# Autodesk Inventor assembly: Protocube
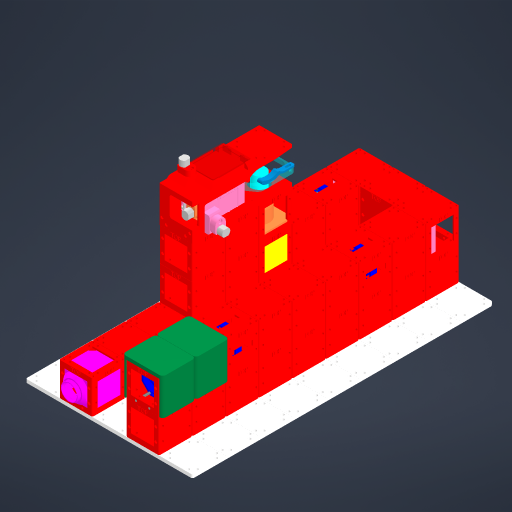
[picture p0: Inventor's stored thumbnail of the model, 512x512]
Saved by Autodesk Inventor 2023.4 (Build 274418000, 418)
## iProperties
Created: 2022-08-13
Part Number: Protocube
Document SubType Name: Assembly
Designer: xSibe
Author: xSibe
## Documents named in this file (12)
- C:\.Laptop\.Work\Projects\Project Protocube\Github\CAD, STL, OBJ Files\1 CAD\Protocube.iam
- C:\.Laptop\.Work\Projects\Project Protocube\1 Autodesk\1 Cubes\Baseplates\Baseplate 9x5 V5.ipt
- C:\.Laptop\.Work\Projects\Project Protocube\1 Autodesk\1 Cubes\Laser\Cube 1x1 V5 (Green Laser).iam
- C:\.Laptop\.Work\Projects\Project Protocube\1 Autodesk\1 Cubes\Lense\Cube 1x1 V5 (Half Inch Lense).iam
- C:\.Laptop\.Work\Projects\Project Protocube\1 Autodesk\1 Cubes\Mirror\Cube 1x1 V5 (Mirror Vertical).iam
- C:\.Laptop\.Work\Projects\Project Protocube\1 Autodesk\1 Cubes\Dichroic\Cube 1x1 V5 (Dichroic).iam
- C:\.Laptop\.Work\Projects\Project Protocube\1 Autodesk\1 Cubes\Objective\Cube 1x1 V5 (Objective).iam
- C:\.Laptop\.Work\Projects\Project Protocube\1 Autodesk\1 Cubes\Camera\Cube 1x1 V5 (Camera).iam
- C:\.Laptop\.Work\Projects\Project Protocube\1 Autodesk\1 Cubes\Mirror\Cube 1x1 V5 (Mirror Horizontal).iam
- C:\.Laptop\.Work\Projects\Project Protocube\1 Autodesk\1 Cubes\Cubes\Cube 1x1 V5 Closed.iam
- C:\.Laptop\.Work\Projects\Project Protocube\1 Autodesk\1 Cubes\Lense\Cube 1x1 V5 (One Inch Lense).iam
- C:\.Laptop\.Work\Projects\Project Protocube\1 Autodesk\1 Cubes\XYZ Stage\XYZ Stage V5.iam
## Components (39 placed, 11 different names)
1. Baseplate 9x5 V5:1 — Mate:27, Mate:46, Mate:47, Mate:48, Mate:52, Mate:53, Mate:60, Mate:61, Mate:62, Mate:65, Mate:66, Mate:67, Mate:69, Mate:70, Mate:71, Mate:93, Mate:94, Mate:95, Mate:98, Mate:99, Mate:100
2. Cube 1x1 V5 (Green Laser):1 [sub-assembly] — Mate:76, Flush:6, Flush:7
3. Cube 1x1 V5 (Mirror Vertical):1 [sub-assembly] — Mate:46, Mate:47, Mate:48, Flush:22, Flush:86, Mate:92
4. Cube 1x1 V5 (Mirror Horizontal):1 [sub-assembly] — Mate:81, Flush:14, Flush:15
5. Cube 1x1 V5 (Mirror Horizontal):2 [sub-assembly] — Flush:16, Flush:17, Mate:82
6. Cube 1x1 V5 (Half Inch Lense):1 [sub-assembly] — Mate:77, Flush:8, Flush:9
7. Cube 1x1 V5 (One Inch Lense):1 [sub-assembly] — Mate:96, Flush:87, Flush:88
8. Cube 1x1 V5 (One Inch Lense):2 [sub-assembly] — Mate:97, Flush:89, Flush:90
9. Cube 1x1 V5 (One Inch Lense):3 [sub-assembly] — Mate:98, Mate:99, Mate:100
10. Cube 1x1 V5 (Dichroic):1 [sub-assembly] — Flush:22, Flush:86, Mate:86, Flush:23, Flush:24, Mate:92
11. Cube 1x1 V5 (Camera):1 [sub-assembly] — Mate:27, Mate:52, Mate:53
12. Cube 1x1 V5 (Objective):1 [sub-assembly] — Mate:86, Flush:23, Flush:24, Mate:101, Mate:102, Mate:103
13. XYZ Stage V5:1 [sub-assembly] — Mate:101, Mate:102, Mate:103
14. Cube 1x1 V5 Closed:13 [sub-assembly] — Flush:3, Mate:80, Flush:13
15. Cube 1x1 V5 Closed:17 [sub-assembly] — Flush:20, Flush:21, Mate:84
16. Cube 1x1 V5 Closed:1 [sub-assembly] — Mate:60, Mate:61, Mate:62, Mate:76, Flush:6, Flush:7
17. Cube 1x1 V5 Closed:2 [sub-assembly]
18. Cube 1x1 V5 Closed:3 [sub-assembly] — Mate:77, Flush:8, Flush:9
19. Cube 1x1 V5 Closed:4 [sub-assembly] — Flush:2, Mate:78, Flush:10
20. Cube 1x1 V5 Closed:5 [sub-assembly]
21. Cube 1x1 V5 Closed:6 [sub-assembly]
22. Cube 1x1 V5 Closed:7 [sub-assembly] — Mate:96, Flush:87, Flush:88
23. Cube 1x1 V5 Closed:8 [sub-assembly] — Flush:3, Mate:80, Flush:13
24. Cube 1x1 V5 Closed:9 [sub-assembly] — Mate:81, Flush:14, Flush:15
25. Cube 1x1 V5 Closed:10 [sub-assembly] — Flush:2, Mate:78, Flush:10
26. Cube 1x1 V5 Closed:11 [sub-assembly]
27. Cube 1x1 V5 Closed:12 [sub-assembly]
28. Cube 1x1 V5 Closed:14 [sub-assembly] — Mate:65, Mate:66, Mate:67, Flush:16, Flush:17, Mate:82
29. Cube 1x1 V5 Closed:15 [sub-assembly] — Mate:97, Flush:89, Flush:90
30. Cube 1x1 V5 Closed:16 [sub-assembly] — Flush:20, Mate:84, Flush:21
31. Cube 1x1 V5 Closed:18 [sub-assembly] — Mate:69, Mate:70, Mate:71, Flush:5, Mate:91, Flush:27
32. Cube 1x1 V5 Closed:19 [sub-assembly]
33. Cube 1x1 V5 Closed:20 [sub-assembly]
34. Cube 1x1 V5 Closed:21 [sub-assembly] — Flush:5, Mate:91, Flush:27
35. Cube 1x1 V5 Closed:22 [sub-assembly]
36. Cube 1x1 V5 Closed:23 [sub-assembly]
37. Cube 1x1 V5 Closed:24 [sub-assembly]
38. Cube 1x1 V5 Closed:25 [sub-assembly] — Mate:93, Mate:94, Mate:95
39. Cube 1x1 V5 Closed:26 [sub-assembly]
## Component patterns: (9 elements, first: Cube 1x1 V5 Closed:1), (3 elements, first: Cube 1x1 V5 Closed:10), (3 elements, first: Cube 1x1 V5 Closed:14), (3 elements, first: Cube 1x1 V5 Closed:18), (4 elements, first: Cube 1x1 V5 Closed:21), (2 elements, first: Cube 1x1 V5 Closed:25)
## Relationships (60: Mate 36, Flush 24)
- Mate:27: Baseplate 9x5 V5:1 ↔ Cube 1x1 V5 (Camera):1
- Mate:46: Baseplate 9x5 V5:1 ↔ Cube 1x1 V5 (Mirror Vertical):1
- Mate:47: Baseplate 9x5 V5:1 ↔ Cube 1x1 V5 (Mirror Vertical):1
- Mate:48: Baseplate 9x5 V5:1 ↔ Cube 1x1 V5 (Mirror Vertical):1
- Mate:52: Baseplate 9x5 V5:1 ↔ Cube 1x1 V5 (Camera):1
- Mate:53: Baseplate 9x5 V5:1 ↔ Cube 1x1 V5 (Camera):1
- Mate:60: Baseplate 9x5 V5:1 ↔ Cube 1x1 V5 Closed:1
- Mate:61: Baseplate 9x5 V5:1 ↔ Cube 1x1 V5 Closed:1
- Mate:62: Baseplate 9x5 V5:1 ↔ Cube 1x1 V5 Closed:1
- Flush:2: Cube 1x1 V5 Closed:4 ↔ Cube 1x1 V5 Closed:10
- Flush:3: Cube 1x1 V5 Closed:13 ↔ Cube 1x1 V5 Closed:8
- Mate:65: Baseplate 9x5 V5:1 ↔ Cube 1x1 V5 Closed:14
- Mate:66: Baseplate 9x5 V5:1 ↔ Cube 1x1 V5 Closed:14
- Mate:67: Baseplate 9x5 V5:1 ↔ Cube 1x1 V5 Closed:14
- Mate:69: Baseplate 9x5 V5:1 ↔ Cube 1x1 V5 Closed:18
- Mate:70: Baseplate 9x5 V5:1 ↔ Cube 1x1 V5 Closed:18
- Mate:71: Baseplate 9x5 V5:1 ↔ Cube 1x1 V5 Closed:18
- Flush:5: Cube 1x1 V5 Closed:18 ↔ Cube 1x1 V5 Closed:21
- Mate:76: Cube 1x1 V5 (Green Laser):1 ↔ Cube 1x1 V5 Closed:1
- Flush:6: Cube 1x1 V5 (Green Laser):1 ↔ Cube 1x1 V5 Closed:1
- Flush:7: Cube 1x1 V5 (Green Laser):1 ↔ Cube 1x1 V5 Closed:1
- Mate:77: Cube 1x1 V5 (Half Inch Lense):1 ↔ Cube 1x1 V5 Closed:3
- Flush:8: Cube 1x1 V5 (Half Inch Lense):1 ↔ Cube 1x1 V5 Closed:3
- Flush:9: Cube 1x1 V5 (Half Inch Lense):1 ↔ Cube 1x1 V5 Closed:3
- Mate:78: Cube 1x1 V5 Closed:4 ↔ Cube 1x1 V5 Closed:10
- Flush:10: Cube 1x1 V5 Closed:4 ↔ Cube 1x1 V5 Closed:10
- Mate:80: Cube 1x1 V5 Closed:13 ↔ Cube 1x1 V5 Closed:8
- Flush:13: Cube 1x1 V5 Closed:13 ↔ Cube 1x1 V5 Closed:8
- Mate:81: Cube 1x1 V5 (Mirror Horizontal):1 ↔ Cube 1x1 V5 Closed:9
- Flush:14: Cube 1x1 V5 (Mirror Horizontal):1 ↔ Cube 1x1 V5 Closed:9
- Flush:15: Cube 1x1 V5 (Mirror Horizontal):1 ↔ Cube 1x1 V5 Closed:9
- Flush:16: Cube 1x1 V5 (Mirror Horizontal):2 ↔ Cube 1x1 V5 Closed:14
- Flush:17: Cube 1x1 V5 (Mirror Horizontal):2 ↔ Cube 1x1 V5 Closed:14
- Mate:82: Cube 1x1 V5 (Mirror Horizontal):2 ↔ Cube 1x1 V5 Closed:14
- Flush:20: Cube 1x1 V5 Closed:17 ↔ Cube 1x1 V5 Closed:16
- Flush:21: Cube 1x1 V5 Closed:17 ↔ Cube 1x1 V5 Closed:16
- Mate:84: Cube 1x1 V5 Closed:17 ↔ Cube 1x1 V5 Closed:16
- Flush:22: Cube 1x1 V5 (Mirror Vertical):1 ↔ Cube 1x1 V5 (Dichroic):1
- Flush:86: Cube 1x1 V5 (Mirror Vertical):1 ↔ Cube 1x1 V5 (Dichroic):1
- Mate:86: Cube 1x1 V5 (Dichroic):1 ↔ Cube 1x1 V5 (Objective):1
- Flush:23: Cube 1x1 V5 (Dichroic):1 ↔ Cube 1x1 V5 (Objective):1
- Flush:24: Cube 1x1 V5 (Dichroic):1 ↔ Cube 1x1 V5 (Objective):1
- Mate:91: Cube 1x1 V5 Closed:18 ↔ Cube 1x1 V5 Closed:21
- Flush:27: Cube 1x1 V5 Closed:18 ↔ Cube 1x1 V5 Closed:21
- Mate:92: Cube 1x1 V5 (Mirror Vertical):1 ↔ Cube 1x1 V5 (Dichroic):1
- Mate:93: Baseplate 9x5 V5:1 ↔ Cube 1x1 V5 Closed:25
- Mate:94: Baseplate 9x5 V5:1 ↔ Cube 1x1 V5 Closed:25
- Mate:95: Baseplate 9x5 V5:1 ↔ Cube 1x1 V5 Closed:25
- Mate:96: Cube 1x1 V5 (One Inch Lense):1 ↔ Cube 1x1 V5 Closed:7
- Flush:87: Cube 1x1 V5 (One Inch Lense):1 ↔ Cube 1x1 V5 Closed:7
- Flush:88: Cube 1x1 V5 (One Inch Lense):1 ↔ Cube 1x1 V5 Closed:7
- Mate:97: Cube 1x1 V5 (One Inch Lense):2 ↔ Cube 1x1 V5 Closed:15
- Flush:89: Cube 1x1 V5 (One Inch Lense):2 ↔ Cube 1x1 V5 Closed:15
- Flush:90: Cube 1x1 V5 (One Inch Lense):2 ↔ Cube 1x1 V5 Closed:15
- Mate:98: Baseplate 9x5 V5:1 ↔ Cube 1x1 V5 (One Inch Lense):3
- Mate:99: Baseplate 9x5 V5:1 ↔ Cube 1x1 V5 (One Inch Lense):3
- Mate:100: Baseplate 9x5 V5:1 ↔ Cube 1x1 V5 (One Inch Lense):3
- Mate:101: Cube 1x1 V5 (Objective):1 ↔ XYZ Stage V5:1
- Mate:102: Cube 1x1 V5 (Objective):1 ↔ XYZ Stage V5:1
- Mate:103: Cube 1x1 V5 (Objective):1 ↔ XYZ Stage V5:1
